# Autodesk Inventor assembly: maze_version2
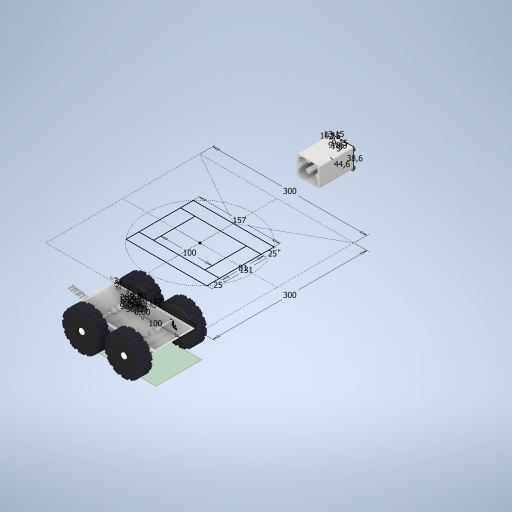
[picture p0: Inventor's stored thumbnail of the model, 512x512]
Saved by Autodesk Inventor 2023 (Build 270158000, 158)
## iProperties
Created: 2026-06-23
Part Number: maze_version2
Document SubType Name: Assembly
Designer: garin
Author: garin
## Documents named in this file (6)
- C:\Users\garin\Documents\Git\Maze-2025\construction\version2\maze_version2.iam
- C:\Users\garin\Documents\base.ipt
- C:\Users\garin\Documents\Git\Maze-2025\construction\version2\DDSM210.ipt
- C:\Users\garin\Documents\Git\Maze-2025\construction\version2\akkum\akkum.iam
- C:\Users\garin\Documents\Git\Maze-2025\construction\version2\akkum\low_part.ipt
- C:\Users\garin\Documents\Git\Maze-2025\construction\version2\screws\hex_screws_M2.5x8mm.ipt
## Components (19 placed, 5 different names)
1. base:1
2. low_part:1 — Заподлицо:1, Заподлицо:2, Заподлицо:3, Совмещение:4, Совмещение:5, Совмещение:6, Совмещение:1, Совмещение:2, Совмещение:3, Совмещение:7, Совмещение:8, Совмещение:9, Совмещение:10, Совмещение:11, Совмещение:12, Заподлицо:4, Совмещение:13, Совмещение:14, Совмещение:15, Совмещение:16, Совмещение:17, Совмещение:18, Совмещение:19, Совмещение:20
3. DDSM210:1 — Совмещение:4, Совмещение:5, Совмещение:6
4. DDSM210:2 — Совмещение:1, Совмещение:2, Совмещение:3
5. DDSM210:3 — Совмещение:10, Совмещение:11, Совмещение:12
6. DDSM210:4 — Совмещение:7, Совмещение:8, Совмещение:9
7. akkum:2 [sub-assembly]
8. hex_screws_M2.5x8mm:1 — Совмещение:13, Совмещение:14
9. hex_screws_M2.5x8mm:2
10. hex_screws_M2.5x8mm:3
11. hex_screws_M2.5x8mm:4 — Совмещение:17, Совмещение:18
12. hex_screws_M2.5x8mm:5 — Совмещение:19, Совмещение:20
13. hex_screws_M2.5x8mm:6
14. hex_screws_M2.5x8mm:7
15. hex_screws_M2.5x8mm:8
16. hex_screws_M2.5x8mm:9
17. hex_screws_M2.5x8mm:10
18. hex_screws_M2.5x8mm:11
19. hex_screws_M2.5x8mm:12 — Совмещение:15, Совмещение:16
## Relationships (24: Mate 20, Flush 4)
- Заподлицо:1 [Flush]: low_part:1
- Заподлицо:2 [Flush]: low_part:1
- Заподлицо:3 [Flush]: low_part:1
- Совмещение:4 [Mate]: low_part:1 ↔ DDSM210:1
- Совмещение:5 [Mate]: low_part:1 ↔ DDSM210:1
- Совмещение:6 [Mate]: low_part:1 ↔ DDSM210:1
- Совмещение:1 [Mate]: low_part:1 ↔ DDSM210:2
- Совмещение:2 [Mate]: low_part:1 ↔ DDSM210:2
- Совмещение:3 [Mate]: low_part:1 ↔ DDSM210:2
- Совмещение:7 [Mate]: low_part:1 ↔ DDSM210:4
- Совмещение:8 [Mate]: low_part:1 ↔ DDSM210:4
- Совмещение:9 [Mate]: low_part:1 ↔ DDSM210:4
- Совмещение:10 [Mate]: low_part:1 ↔ DDSM210:3
- Совмещение:11 [Mate]: low_part:1 ↔ DDSM210:3
- Совмещение:12 [Mate]: low_part:1 ↔ DDSM210:3
- Заподлицо:4 [Flush] (23 mm): low_part:1
- Совмещение:13 [Mate]: low_part:1 ↔ hex_screws_M2.5x8mm:1
- Совмещение:14 [Mate]: low_part:1 ↔ hex_screws_M2.5x8mm:1
- Совмещение:15 [Mate]: low_part:1 ↔ hex_screws_M2.5x8mm:12
- Совмещение:16 [Mate]: low_part:1 ↔ hex_screws_M2.5x8mm:12
- Совмещение:17 [Mate]: low_part:1 ↔ hex_screws_M2.5x8mm:4
- Совмещение:18 [Mate]: low_part:1 ↔ hex_screws_M2.5x8mm:4
- Совмещение:19 [Mate]: low_part:1 ↔ hex_screws_M2.5x8mm:5
- Совмещение:20 [Mate]: low_part:1 ↔ hex_screws_M2.5x8mm:5
